# Autodesk Inventor assembly: Assembly1
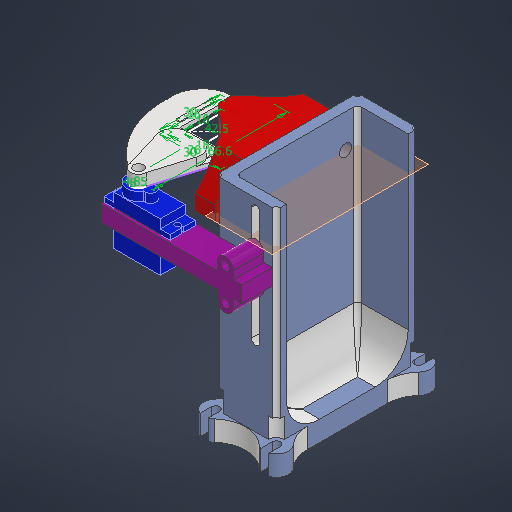
[picture p0: Inventor's stored thumbnail of the model, 512x512]
Saved by Autodesk Inventor 2025.1 (Build 291241000, 241)
## iProperties
Created: 2025-02-14
Part Number: Assembly1
Document SubType Name: Assembly
Designer: m_kni
Author: m_kni
## Documents named in this file (6)
- C:\Users\jerem\Documents\GitHub\Perovskite-Automated-Synthesis-System\CAD\Spectrometer_Mount\Assembly1.iam
- C:\Users\jerem\Documents\GitHub\Perovskite-Automated-Synthesis-System\CAD\Spectrometer_Mount\Infeed_Tower.ipt
- C:\Users\jerem\Documents\GitHub\Perovskite-Automated-Synthesis-System\CAD\Spectrometer_Mount\servo_holder.ipt
- C:\Users\jerem\Documents\GitHub\Perovskite-Automated-Synthesis-System\CAD\Non 3D Printed Parts\Motors and Servos\SG90 Servo.ipt
- C:\Users\jerem\Documents\GitHub\Perovskite-Automated-Synthesis-System\CAD\Spectrometer_Mount\scanner.ipt
- C:\Users\jerem\Documents\GitHub\Perovskite-Automated-Synthesis-System\CAD\Spectrometer_Mount\infeed plate.ipt
## Components (5 placed, 5 different names)
1. Infeed_Tower:1 — Mate:1, Flush:1, Flush:2, Insert:2
2. servo_holder:1 — Mate:1, Flush:1, Flush:2, Insert:1, Angle:1
3. SG90 Servo:1 — Insert:1, Angle:1, Insert:3
4. scanner:1 — Insert:2
5. infeed plate:1 — Insert:3
## Relationships (7: Insert 3, Flush 2, Mate 1, Angle 1)
- Mate:1: Infeed_Tower:1 ↔ servo_holder:1
- Flush:1 (-25.5 mm): Infeed_Tower:1 ↔ servo_holder:1
- Flush:2 (-13.5 mm): Infeed_Tower:1 ↔ servo_holder:1
- Insert:1: servo_holder:1 ↔ SG90 Servo:1
- Angle:1 (90 deg): servo_holder:1 ↔ SG90 Servo:1
- Insert:2: Infeed_Tower:1 ↔ scanner:1
- Insert:3: SG90 Servo:1 ↔ infeed plate:1
